# Autodesk Inventor assembly: Epsilon gripper 2
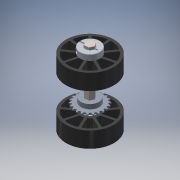
[picture p0: Inventor's stored thumbnail of the model, 180x180]
Saved by Autodesk Inventor 2019 (Build 230136000, 136)
## iProperties
Created: 2019-02-08
Part Number: Epsilon gripper 2
Document SubType Name: Assembly
Designer: josh
Author: josh
## Documents named in this file (6)
- D:\Synthesis Robots\Epsilon\Epsilon Grabbers\Grabbing unit\Epsilon gripper 2.iam
- D:\Synthesis Robots\Epsilon\Epsilon Grabbers\Grabbing unit\am-0856 500 Hex Shaft for Modulox REV3.ipt
- D:\Synthesis Robots\Epsilon\Epsilon Grabbers\am-0646 S25-22HA-500 Hex Sprocket.ipt
- D:\Synthesis Robots\Epsilon\Epsilon Grabbers\am-3946 3IN 500Hex Molded Compliant Wheel VER 2.ipt
- D:\Synthesis Robots\Epsilon\Epsilon Grabbers\am-0864 Hex Spacer for Modulox.ipt
- D:\Synthesis Robots\Epsilon\Epsilon Grabbers\am-1238 Collar Clamp, 0.5'' Hex Bore, Aluminum REV2.iam
## Components (8 placed, 5 different names)
1. am-0856 500 Hex Shaft for Modulox REV3:1 — Mate:14, Mate:15, Mate:16, Mate:17
2. am-0646 S25-22HA-500 Hex Sprocket:1
3. am-3946 3IN 500Hex Molded Compliant Wheel VER 2:1 — Mate:19
4. am-3946 3IN 500Hex Molded Compliant Wheel VER 2:2 — Mate:18
5. am-0864 Hex Spacer for Modulox:1
6. am-0864 Hex Spacer for Modulox:2
7. am-1238 Collar Clamp, 0.5'' Hex Bore, Aluminum REV2:1 [sub-assembly] — Mate:14, Mate:15, Mate:19
8. am-1238 Collar Clamp, 0.5'' Hex Bore, Aluminum REV2:2 [sub-assembly] — Mate:16, Mate:17, Mate:18
## Relationships (19: Mate 19)
- [Mate]: am-0856 500 Hex Shaft for Modulox REV3:1 ↔ am-3946 3IN 500Hex Molded Compliant Wheel VER 2:1
- [Mate]: am-0856 500 Hex Shaft for Modulox REV3:1 ↔ am-3946 3IN 500Hex Molded Compliant Wheel VER 2:1
- [Mate]: am-0856 500 Hex Shaft for Modulox REV3:1 ↔ am-0646 S25-22HA-500 Hex Sprocket:1
- [Mate]: am-0856 500 Hex Shaft for Modulox REV3:1 ↔ am-0646 S25-22HA-500 Hex Sprocket:1
- [Mate]: am-0856 500 Hex Shaft for Modulox REV3:1 ↔ am-0864 Hex Spacer for Modulox:2
- [Mate]: am-0856 500 Hex Shaft for Modulox REV3:1 ↔ am-0864 Hex Spacer for Modulox:2
- [Mate]: am-3946 3IN 500Hex Molded Compliant Wheel VER 2:1 ↔ am-0864 Hex Spacer for Modulox:2
- [Mate]: am-0856 500 Hex Shaft for Modulox REV3:1 ↔ am-0864 Hex Spacer for Modulox:1
- [Mate]: am-0856 500 Hex Shaft for Modulox REV3:1 ↔ am-0864 Hex Spacer for Modulox:1
- [Mate]: am-0646 S25-22HA-500 Hex Sprocket:1 ↔ am-0864 Hex Spacer for Modulox:1
- [Mate]: am-0856 500 Hex Shaft for Modulox REV3:1 ↔ am-3946 3IN 500Hex Molded Compliant Wheel VER 2:2
- [Mate]: am-0856 500 Hex Shaft for Modulox REV3:1 ↔ am-3946 3IN 500Hex Molded Compliant Wheel VER 2:2
- [Mate]: am-3946 3IN 500Hex Molded Compliant Wheel VER 2:2 ↔ am-0864 Hex Spacer for Modulox:1
- Mate:14: am-0856 500 Hex Shaft for Modulox REV3:1 ↔ am-1238 Collar Clamp, 0.5'' Hex Bore, Aluminum REV2:1
- Mate:15: am-0856 500 Hex Shaft for Modulox REV3:1 ↔ am-1238 Collar Clamp, 0.5'' Hex Bore, Aluminum REV2:1
- Mate:16: am-0856 500 Hex Shaft for Modulox REV3:1 ↔ am-1238 Collar Clamp, 0.5'' Hex Bore, Aluminum REV2:2
- Mate:17: am-0856 500 Hex Shaft for Modulox REV3:1 ↔ am-1238 Collar Clamp, 0.5'' Hex Bore, Aluminum REV2:2
- Mate:18: am-3946 3IN 500Hex Molded Compliant Wheel VER 2:2 ↔ am-1238 Collar Clamp, 0.5'' Hex Bore, Aluminum REV2:2
- Mate:19: am-3946 3IN 500Hex Molded Compliant Wheel VER 2:1 ↔ am-1238 Collar Clamp, 0.5'' Hex Bore, Aluminum REV2:1
